# Autodesk Inventor assembly: Assembled
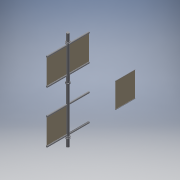
[picture p0: Inventor's stored thumbnail of the model, 180x180]
Saved by Autodesk Inventor 2016 SP1 (Build 200210100, 210)
## iProperties
Created: 2016-07-02
Part Number: Assembled
Document SubType Name: Assembly
Designer: Tore Den Store
Author: Tore Den Store
## Documents named in this file (3)
- C:\Users\Jonatan\Documents\Inventor\Vertical axis wind turbine\1 of 4 part\Assembled.iam
- C:\Users\Jonatan\Documents\Inventor\Vertical axis wind turbine\1 of 4 part\CentralBeam.ipt
- C:\Users\Jonatan\Documents\Inventor\Vertical axis wind turbine\1 of 4 part\Sail.ipt
## Components (5 placed, 2 different names)
1. CentralBeam:1 — Rigid:1, Rigid:2, Rigid:3
2. Sail:1 — Rigid:1
3. Sail:2 — Rigid:3
4. Sail:3
5. Sail:4 — Rigid:2
## Relationships (3: WeldJoint 3)
- Rigid:1 [WeldJoint]: CentralBeam:1 ↔ Sail:1
- Rigid:2 [WeldJoint]: CentralBeam:1 ↔ Sail:4
- Rigid:3 [WeldJoint]: CentralBeam:1 ↔ Sail:2
